# Autodesk Inventor assembly: gears_MIR
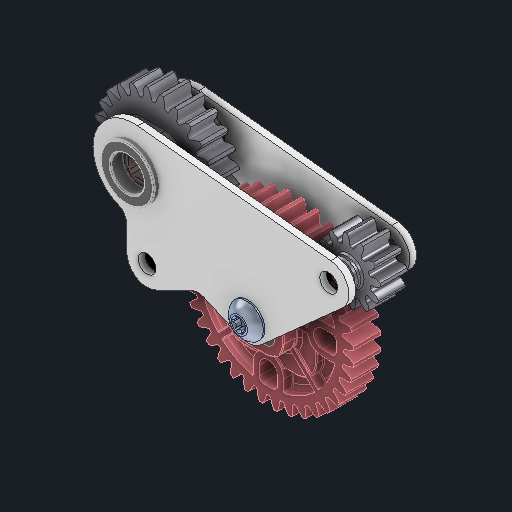
[picture p0: Inventor's stored thumbnail of the model, 512x512]
Saved by Autodesk Inventor 2024 (Build 280153000, 153)
## iProperties
Created: 2023-08-16
Part Number: gears_MIR
Document SubType Name: Assembly
Designer: avere
Author: avere
## Documents named in this file (12)
- D:\vex_robotics\hardware\cad\scrap_v0.1\catapult\mirrored_parts\gears_MIR.iam
- D:\vex_robotics\hardware\cad\scrap_v0.1\catapult\mirrored_parts\gear_gusset_MIR.ipt
- D:\vex_robotics\hardware\cad\scrap_v0.1\catapult\mirrored_parts\HS Bushing 0.1250_MIR.ipt
- D:\vex_robotics\hardware\cad\scrap_v0.1\catapult\mirrored_parts\half_cut_24_MIR.ipt
- D:\vex_robotics\hardware\cad\scrap_v0.1\catapult\mirrored_parts\LS 12T Gear Steel_MIR.ipt
- D:\vex_robotics\hardware\cad\VEX-CAD-Inventor-1.41\Structure\Hardware\Screw Steel - Star\SScrew Star Smooth .750.ipt
- D:\vex_robotics\hardware\cad\VEX-CAD-Inventor-1.41\Structure\Hardware\Nut Nylon\Nut Nylon - White.ipt
- D:\vex_robotics\hardware\cad\scrap_v0.1\catapult\custom_parts\half_cut_36t.ipt
- D:\vex_robotics\hardware\cad\VEX-CAD-Inventor-1.41\Structure\Standoff\Standoff .50.ipt
- D:\cad\VEX-CAD-Inventor-1.41\Structure\Hardware\Screw Steel - Star.ipt
- D:\cad\VEX-CAD-Inventor-1.41\Structure\Hardware\Nut Nylon.ipt
- D:\cad\VEX-CAD-Inventor-1.41\Structure\Standoff.ipt
## Components (10 placed, 8 different names)
1. gear_gusset_MIR:1 — Insert:1, Insert:5, Insert:7, Insert:9
2. HS Bushing 0.1250_MIR:1 — Insert:1, Insert:4
3. gear_gusset_MIR:2 — Insert:2, Insert:6, Insert:8
4. HS Bushing 0.1250_MIR:2 — Insert:2
5. half_cut_24_MIR:1 — Insert:4
6. LS 12T Gear Steel_MIR:1 — Insert:8
7. SScrew Star Smooth .750:1 — Insert:5
8. Nut Nylon - White:1 — Insert:6
9. half_cut_36t:1 — Insert:7
10. Standoff .50:1 — Insert:9
## Relationships (8: Insert 8)
- Insert:1: gear_gusset_MIR:1 ↔ HS Bushing 0.1250_MIR:1
- Insert:2: gear_gusset_MIR:2 ↔ HS Bushing 0.1250_MIR:2
- Insert:4: HS Bushing 0.1250_MIR:1 ↔ half_cut_24_MIR:1
- Insert:5: gear_gusset_MIR:1 ↔ SScrew Star Smooth .750:1
- Insert:6: gear_gusset_MIR:2 ↔ Nut Nylon - White:1
- Insert:7: gear_gusset_MIR:1 ↔ half_cut_36t:1
- Insert:8 (1.5875 mm): gear_gusset_MIR:2 ↔ LS 12T Gear Steel_MIR:1
- Insert:9: gear_gusset_MIR:1 ↔ Standoff .50:1
